# Autodesk Inventor assembly: дрон сборка
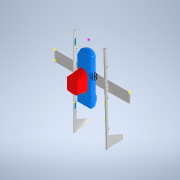
[picture p0: Inventor's stored thumbnail of the model, 180x180]
Saved by Autodesk Inventor 2022 (Build 260153000, 153)
## iProperties
Created: 2021-12-25
Part Number: дрон сборка
Document SubType Name: Assembly
Designer: Grigori
Author: Grigori
## Documents named in this file (4)
- C:\Users\User\Documents\GitHub\ModularDrone\Сборка1\дрон сборка общая.iam
- C:\Users\User\Documents\GitHub\ModularDrone\Сборка1\Сборка крышка.iam
- C:\Users\User\Documents\GitHub\ModularDrone\Сборка1\корпус.ipt
- C:\Users\User\Documents\GitHub\ModularDrone\PartsModels\корбка\коробка корпус 3.ipt
## Components (3 placed, 3 different names)
1. Сборка крышка:1 [sub-assembly] — Вставка:1
2. корпус:1 — Вставка:1, Совмещение:1
3. коробка корпус 3:1 — Совмещение:1
## Relationships (2: Insert 1, Mate 1)
- Вставка:1 [Insert]: Сборка крышка:1 ↔ корпус:1
- Совмещение:1 [Mate]: корпус:1 ↔ коробка корпус 3:1
